# Autodesk Inventor assembly: 02_Bark
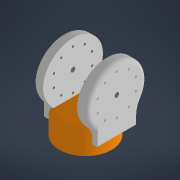
[picture p0: Inventor's stored thumbnail of the model, 180x180]
Saved by Autodesk Inventor 2022 (Build 260153000, 153)
## iProperties
Created: 2022-05-07
Part Number: 02_Bark
Document SubType Name: Assembly
Designer: pzach
Author: pzach
## Documents named in this file (4)
- D:\GIT\Studia\Semestr4\MiSR\Robot\02_Bark.iam
- D:\GIT\Studia\Semestr4\MiSR\Robot\02_DoF1_Podstawa.ipt
- D:\GIT\Studia\Semestr4\MiSR\Robot\03_DoF1_Bark.ipt
- D:\GIT\Studia\Semestr4\MiSR\Robot\03_DoF1_Bark_MIR2.ipt
## Components (3 placed, 3 different names)
1. 02_DoF1_Podstawa:1 — Mate:3, Mate:4, Mate:5, Angle:1, Mate:6, Mate:7, Mate:8
2. 03_DoF1_Bark:1 — Mate:3, Mate:4, Mate:5
3. 03_DoF1_Bark_MIR2:1 — Angle:1, Mate:6, Mate:7, Mate:8
## Relationships (7: Mate 6, Angle 1)
- Mate:3: 02_DoF1_Podstawa:1 ↔ 03_DoF1_Bark:1
- Mate:4: 02_DoF1_Podstawa:1 ↔ 03_DoF1_Bark:1
- Mate:5: 02_DoF1_Podstawa:1 ↔ 03_DoF1_Bark:1
- Angle:1 (0 deg): 02_DoF1_Podstawa:1 ↔ 03_DoF1_Bark_MIR2:1
- Mate:6: 02_DoF1_Podstawa:1 ↔ 03_DoF1_Bark_MIR2:1
- Mate:7: 02_DoF1_Podstawa:1 ↔ 03_DoF1_Bark_MIR2:1
- Mate:8: 02_DoF1_Podstawa:1 ↔ 03_DoF1_Bark_MIR2:1
